# Autodesk Inventor assembly: new_assembly_auger
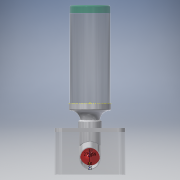
[picture p0: Inventor's stored thumbnail of the model, 180x180]
Saved by Autodesk Inventor 2019 (Build 230136000, 136)
## iProperties
Created: 2019-01-23
Part Number: new_assembly_auger
Document SubType Name: Assembly
Designer: jmc
Author: jmc
## Documents named in this file (5)
- D:\Inventor\Projects\CatFeeder\version4 (auger)\new_assembly_auger.iam
- D:\Inventor\Projects\CatFeeder\Case\version3\case_top.ipt
- D:\Inventor\Projects\CatFeeder\Case\version3\case_bottom.ipt
- D:\Inventor\Projects\CatFeeder\version4 (auger)\subassembly_jar_jarcone.iam
- D:\Inventor\Projects\CatFeeder\version4 (auger)\subassembly_auger_case.iam
## Components (4 placed, 4 different names)
1. subassembly_jar_jarcone:1 [sub-assembly] — Rigid:2
2. subassembly_auger_case:1 [sub-assembly] — Rigid:3
3. case_top:1 — Rigid:1, Rigid:2, Rigid:3
4. case_bottom:1 — Rigid:1
## Relationships (3: WeldJoint 3)
- Rigid:1 [WeldJoint]: case_top:1 ↔ case_bottom:1
- Rigid:2 [WeldJoint]: subassembly_jar_jarcone:1 ↔ case_top:1
- Rigid:3 [WeldJoint]: subassembly_auger_case:1 ↔ case_top:1
